# Autodesk Inventor assembly: sunon_fan_red
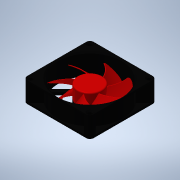
[picture p0: Inventor's stored thumbnail of the model, 180x180]
Saved by Autodesk Inventor 2022 (Build 260153000, 153)
## iProperties
Created: 2015-03-08
Part Number: sunon_fan_red
Document SubType Name: Assembly
Designer: Venci
Author: Venci
## Documents named in this file (3)
- C:\Autodesk\Elementy\fan_80x80\fan_80x80.iam
- C:\Autodesk\Elementy\fan_80x80\sunon_frame (1).ipt
- C:\Autodesk\Elementy\fan_80x80\sunon_blade_80 (1).ipt
## Components (2 placed, 2 different names)
1. sunon_frame (1):1 — Insert:1
2. sunon_blade_80 (1):1 — Insert:1
## Relationships (1: Insert 1)
- Insert:1: sunon_frame (1):1 ↔ sunon_blade_80 (1):1
